# Autodesk Inventor assembly: bellows_kihon
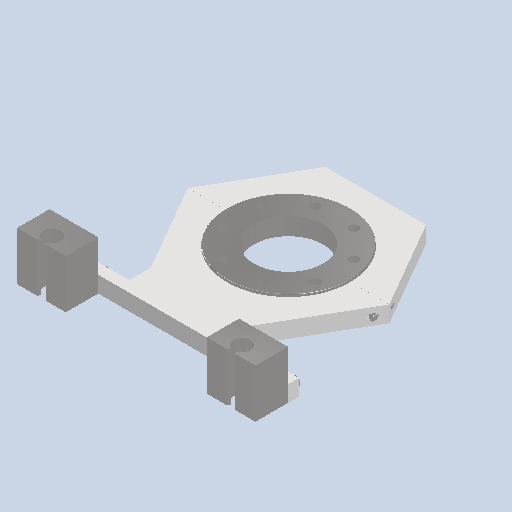
[picture p0: Inventor's stored thumbnail of the model, 512x512]
Saved by Autodesk Inventor 2026.3 (Build 303398000, 398)
## iProperties
Created: 2026-06-03
Part Number: bellows_kihon
Document SubType Name: Assembly
Designer: shusu
Author: shusu
## Documents named in this file (7)
- C:\Users\shusu\aklab_pihti\PIHTI\bellows\bellows_1.iam
- C:\Users\shusu\aklab_pihti\PIHTI\bellows\bellows_flange.ipt
- C:\Users\shusu\aklab_pihti\PIHTI\bellows\flangeclamp_down.ipt
- C:\Users\shusu\aklab_pihti\PIHTI\bellows\flangeclamp_up.ipt
- C:\Users\shusu\OneDrive - Kyoto University\ドキュメント\Inventor\Content Center Files\R2026\ja-JP\JIS B 1176\JIS B 1176 - M3 x 16 - 0.5.ipt
- C:\Users\shusu\aklab_pihti\PIHTI\bellows\linearbearing.ipt
- C:\Users\shusu\OneDrive - Kyoto University\ドキュメント\Inventor\Content Center Files\R2026\ja-JP\JIS B 1176\JIS B 1176 - M5 x 16 - 0.8.ipt
## Components (11 placed, 6 different names)
1. bellows_flange:2 — 挿入:4
2. flangeclamp_down:3 — 挿入:4, 挿入:10, メイト:6, メイト:8, 挿入:13, 挿入:14, 挿入:17, 挿入:18
3. flangeclamp_up:3 — 挿入:8
4. JIS B 1176 - メートル M3 x 16:4 — 挿入:8
5. JIS B 1176 - メートル M3 x 16:6 — 挿入:10
6. linearbearing:2 — メイト:8
7. linearbearing:3 — メイト:6
8. JIS B 1176 - メートル M5 x 16:3 — 挿入:13
9. JIS B 1176 - メートル M5 x 16:4 — 挿入:14
10. JIS B 1176 - メートル M5 x 16:7 — 挿入:18
11. JIS B 1176 - メートル M5 x 16:8 — 挿入:17
## Relationships (11: Insert 7, Mate 4)
- [Mate]: flangeclamp_down:3 ↔ flangeclamp_up:3
- [Mate]: flangeclamp_down:3 ↔ flangeclamp_up:3
- 挿入:4 [Insert] (-15 mm): bellows_flange:2 ↔ flangeclamp_down:3
- 挿入:8 [Insert]: flangeclamp_up:3 ↔ JIS B 1176 - メートル M3 x 16:4
- 挿入:10 [Insert]: flangeclamp_down:3 ↔ JIS B 1176 - メートル M3 x 16:6
- メイト:6 [Mate]: flangeclamp_down:3 ↔ linearbearing:3
- メイト:8 [Mate]: flangeclamp_down:3 ↔ linearbearing:2
- 挿入:13 [Insert]: flangeclamp_down:3 ↔ JIS B 1176 - メートル M5 x 16:3
- 挿入:14 [Insert]: flangeclamp_down:3 ↔ JIS B 1176 - メートル M5 x 16:4
- 挿入:17 [Insert]: flangeclamp_down:3 ↔ JIS B 1176 - メートル M5 x 16:8
- 挿入:18 [Insert]: flangeclamp_down:3 ↔ JIS B 1176 - メートル M5 x 16:7
## Named parameters: d13_d11 = 0 mm, d14_d12 = 0 mm
